# Autodesk Inventor assembly: jig_lineup
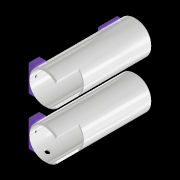
[picture p0: Inventor's stored thumbnail of the model, 180x180]
Saved by Autodesk Inventor 2020.2 (Build 242310000, 310)
## iProperties
Created: 2020-04-29
Part Number: jig_lineup
Document SubType Name: Assembly
Designer: agmlego
Mass: 8782.75 g
Surface Area: 19769.4 cm^2
Volume: 9426.01 cm^3
Density: 0.931757 g/cm^3
Author: agmlego
## Documents named in this file (8)
- D:\syncthing\rwsir-rc7py\projects\CreekFleet\CreekFleet_AutoBuoy\Mechanical CAD\router_jigs\jig_lineup.iam
- D:\syncthing\rwsir-rc7py\projects\CreekFleet\CreekFleet_AutoBuoy\Mechanical CAD\hull\left_hull_mid.ipt
- D:\syncthing\rwsir-rc7py\projects\CreekFleet\CreekFleet_AutoBuoy\Mechanical CAD\hull\right_hull_mid.ipt
- D:\syncthing\rwsir-rc7py\projects\CreekFleet\CreekFleet_AutoBuoy\Mechanical CAD\router_jigs\piercing_flats.ipt
- D:\syncthing\rwsir-rc7py\projects\CreekFleet\CreekFleet_AutoBuoy\Mechanical CAD\router_jigs\aft_holes.ipt
- D:\syncthing\rwsir-rc7py\projects\CreekFleet\CreekFleet_AutoBuoy\Mechanical CAD\router_jigs\controls_flat.ipt
- D:\syncthing\rwsir-rc7py\projects\CreekFleet\CreekFleet_AutoBuoy\Mechanical CAD\router_jigs\strut_hole.ipt
- D:\syncthing\rwsir-rc7py\projects\CreekFleet\CreekFleet_AutoBuoy\Mechanical CAD\router_jigs\controls_holes.ipt
## Components (12 placed, 7 different names)
1. left_hull_mid:1 — Mate:1, Mate:4, Angle:1, Flush:1, Tangent:1, Flush:2, Insert:2, Mate:5, Mate:7, Mate:8, Angle:3, Mate:11, Mate:15, Mate:16, Tangent:3, Mate:18, Angle:4, Mate:19, Insert:3
2. right_hull_mid:1 — Mate:2, Mate:3, Angle:2, Flush:1, Tangent:1, Flush:2, Insert:1, Mate:6, Mate:12, Mate:14, Tangent:2, Mate:17, Angle:5
3. controls_holes:1 — Mate:19, Insert:3
4. piercing_flats:1 — Mate:2, Mate:3, Angle:2, Mate:13
5. piercing_flats:2 — Mate:1, Mate:4, Angle:1
6. controls_flat:1 — Mate:7, Mate:8, Angle:3
7. aft_holes:1 — Insert:2, Mate:5
8. aft_holes:2 — Insert:1, Mate:6
9. strut_hole:1 — Flush:3, Mate:9, Mate:15
10. strut_hole:2 — Flush:4, Mate:10, Mate:14, Angle:5
11. strut_hole:3 — Flush:4, Mate:10, Mate:12, Mate:13
12. strut_hole:4 — Flush:3, Mate:9, Mate:11, Mate:16, Angle:4
## Relationships (34: Mate 19, Angle 5, Flush 4, Tangent 3, Insert 3)
- Mate:1: left_hull_mid:1 ↔ piercing_flats:2
- Mate:2: right_hull_mid:1 ↔ piercing_flats:1
- Mate:3: right_hull_mid:1 ↔ piercing_flats:1
- Mate:4: left_hull_mid:1 ↔ piercing_flats:2
- Angle:1 (0 deg): left_hull_mid:1 ↔ piercing_flats:2
- Angle:2 (0 deg): right_hull_mid:1 ↔ piercing_flats:1
- Flush:1: left_hull_mid:1 ↔ right_hull_mid:1
- Tangent:1 (100 mm): left_hull_mid:1 ↔ right_hull_mid:1
- Flush:2: left_hull_mid:1 ↔ right_hull_mid:1
- Insert:1: right_hull_mid:1 ↔ aft_holes:2
- Insert:2: left_hull_mid:1 ↔ aft_holes:1
- Mate:5: left_hull_mid:1 ↔ aft_holes:1
- Mate:6: right_hull_mid:1 ↔ aft_holes:2
- Mate:7: left_hull_mid:1 ↔ controls_flat:1
- Mate:8: left_hull_mid:1 ↔ controls_flat:1
- Angle:3 (0 deg): left_hull_mid:1 ↔ controls_flat:1
- Flush:3: strut_hole:1 ↔ strut_hole:4
- Flush:4: strut_hole:2 ↔ strut_hole:3
- Mate:9: strut_hole:1 ↔ strut_hole:4
- Mate:10: strut_hole:2 ↔ strut_hole:3
- Mate:11: left_hull_mid:1 ↔ strut_hole:4
- Mate:12: right_hull_mid:1 ↔ strut_hole:3
- Mate:13: piercing_flats:1 ↔ strut_hole:3
- Mate:14: right_hull_mid:1 ↔ strut_hole:2
- Mate:15: left_hull_mid:1 ↔ strut_hole:1
- Mate:16: left_hull_mid:1 ↔ strut_hole:4
- Tangent:2: right_hull_mid:1
- Tangent:3: left_hull_mid:1
- Mate:17: right_hull_mid:1
- Mate:18: left_hull_mid:1
- Angle:4 (180 deg): left_hull_mid:1 ↔ strut_hole:4
- Angle:5 (0 deg): right_hull_mid:1 ↔ strut_hole:2
- Mate:19: left_hull_mid:1 ↔ controls_holes:1
- Insert:3: left_hull_mid:1 ↔ controls_holes:1
